# Autodesk Inventor assembly: !drive-pod-back-left
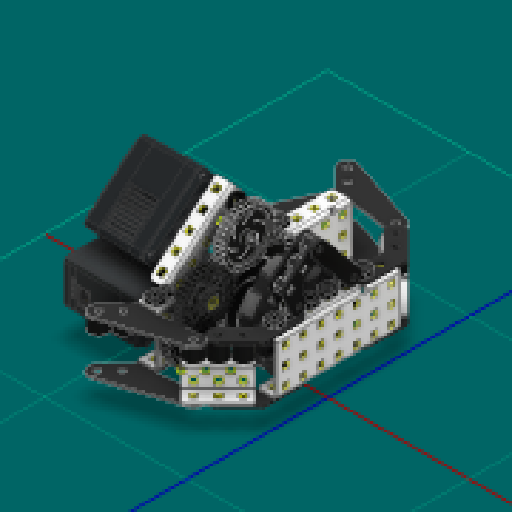
[picture p0: Inventor's stored thumbnail of the model, 512x512]
Saved by Autodesk Inventor 2025 (Build 290162000, 162)
## iProperties
Created: 2024-08-10
Part Number: !drive-pod-back-left
Document SubType Name: Assembly
Designer: averey
Author: averey
## Documents named in this file (25)
- C:\Users\avere\rbp_cad\atlas\chassis\drive-pod-back-left\!drive-pod-back-left.iam
- C:\Users\avere\rbp_cad\atlas\chassis\drive-pod-back-left\LS Pillow Bearing Block-back-left.ipt
- C:\Users\avere\rbp_cad\atlas\chassis\drive-pod-back-left\gearbox-support-gusset-back-left.ipt
- C:\Users\avere\rbp_cad\atlas\chassis\drive-pod-back-left\gearbox-gusset-back-left.ipt
- C:\Users\avere\rbp_cad\atlas\chassis\drive-pod-back-left\Bearing Flat Low Profile-back-left.ipt
- C:\Users\avere\rbp_cad\atlas\chassis\drive-pod-back-left\Alu Angle 1x1x5-back-left.ipt
- C:\Users\avere\rbp_cad\atlas\chassis\drive-pod-back-left\SteelM-StarS-back-left.iam
- C:\Users\avere\rbp_cad\atlas\chassis\drive-pod-back-left\V5 Motor (5.5W)-back-left.ipt
- C:\Users\avere\rbp_cad\atlas\chassis\drive-pod-back-left\LS 36T Gear-back-left.ipt
- C:\Users\avere\rbp_cad\atlas\chassis\drive-pod-back-left\LS 60T Gear-back-left.ipt
- C:\Users\avere\rbp_cad\atlas\chassis\drive-pod-back-left\2.75 Omni AS, No Insert-back-left.iam
- C:\Users\avere\rbp_cad\atlas\chassis\drive-pod-back-left\LS 12T Gear-back-left.ipt
- C:\Users\avere\rbp_cad\atlas\chassis\drive-pod-back-left\half_cut_36t-back-left.ipt
- C:\Users\avere\rbp_cad\atlas\chassis\drive-pod-back-left\elbow-gusset-back-left.ipt
- C:\Users\avere\rbp_cad\atlas\chassis\drive-pod-back-left\Alu C 1x2x1x3-back-left.ipt
- C:\Users\avere\rbp_cad\atlas\chassis\drive-pod-back-left\join-gusset_offset-back-left.ipt
- C:\Users\avere\rbp_cad\VEX-CAD-Inventor-1.41\Motion\Spacers\Spacer Nylon .500 OD\NSpacer Black .500 OD x .500.ipt
- C:\Users\avere\rbp_cad\VEX-CAD-Inventor-1.41\Motion\Spacers\Spacer Nylon .500 OD.ipt
- C:\Users\avere\rbp_cad\VEX-CAD-Inventor-1.41\Motion\Spacers\Spacer Nylon .500 OD\NSpacer Black .500 OD x .375.ipt
- C:\Users\avere\rbp_cad\VEX-CAD-Inventor-1.41\Structure\C Channel\Aluminum 1x3x1\Alu C 1x3x1x7.ipt
- C:\Users\avere\rbp_cad\VEX-CAD-Inventor-1.41\Structure\C Channel\Aluminum 1x3x1\Alu C 1x3x1x11.ipt
- C:\Users\avere\rbp_cad\atlas\chassis\drive-pod-back-right\join-gusset_offset-back-left-back-right.ipt
- C:\Users\avere\rbp_cad\VEX-CAD-Inventor-1.41\Structure\Standoff\Standoff 1.25.ipt
- C:\Users\avere\rbp_cad\VEX-CAD-Inventor-1.41\Motion\Spacers\Spacer Nylon .375 OD\NSpacer .375 OD x .125.ipt
- C:\Users\avere\rbp_cad\VEX-CAD-Inventor-1.41\Motion\Spacers\Spacer Nylon .375 OD.ipt
## Components (44 placed, 22 different names)
1. LS Pillow Bearing Block-back-left:1 — Mate:7, Insert:11
2. LS Pillow Bearing Block-back-left:2 — Insert:9, Mate:8
3. gearbox-support-gusset-back-left:1 — Insert:9
4. gearbox-gusset-back-left:1 — Mate:7, Mate:9
5. gearbox-support-gusset-back-left:2 — Mate:8
6. gearbox-gusset-back-left:2 — Insert:11
7. Bearing Flat Low Profile-back-left:1 — Mate:9
8. LS Pillow Bearing Block-back-left:3 — Insert:17, Insert:18
9. LS Pillow Bearing Block-back-left:4 — Insert:16
10. Alu Angle 1x1x5-back-left:1 — Insert:16, Mate:12, Mate:13, Mate:22, Insert:31, Insert:30, Insert:32
11. gearbox-gusset-back-left:3 — Mate:12, Insert:17
12. gearbox-gusset-back-left:4 — Mate:13, Insert:18
13. SteelM-StarS-back-left:1 [sub-assembly] — Insert:51, Mate:33
14. V5 Motor (5.5W)-back-left:1 — Mate:22, Insert:31
15. LS 36T Gear-back-left:1 — Insert:29
16. LS 60T Gear-back-left:1 — Insert:28, Mate:21, Insert:53
17. 2.75 Omni AS, No Insert-back-left:1 [sub-assembly] — Insert:28, Mate:21
18. LS 12T Gear-back-left:1 — Insert:29
19. half_cut_36t-back-left:1 — Insert:30
20. LS 36T Gear-back-left:2 — Insert:32
21. elbow-gusset-back-left:1 — Mate:25, Insert:35, Insert:45, Mate:28
22. Alu C 1x2x1x3-back-left:1 — Mate:25, Insert:35, Insert:38, Insert:41
23. elbow-gusset-back-left:2 — Insert:39, Insert:40
24. join-gusset_offset-back-left:1 — Insert:43, Insert:46
25. join-gusset_offset-back-left:2 — Insert:38, Insert:50, Mate:32
26. NSpacer Black .500 OD x .500:1 — Insert:39
27. NSpacer Black .500 OD x .500:2 — Insert:40
28. NSpacer Black .500 OD x .375:3 — Insert:41
29. NSpacer Black .500 OD x .375:4 — Insert:43
30. NSpacer Black .500 OD x .375:5 — Insert:46
31. Alu C 1x2x1x3-back-left:2 — Insert:39, Mate:25, Insert:41, Insert:42, Insert:54, Insert:55
32. elbow-gusset-back-left:3 — Insert:39, Mate:25, Insert:47, Mate:30
33. NSpacer Black .500 OD x .500:6 — Insert:41
34. NSpacer Black .500 OD x .500:7 — Insert:42
35. elbow-gusset-back-left:4 — Insert:48, Mate:29
36. Alu C 1x3x1x7:1 — Insert:45, Mate:28, Insert:47, Insert:48, Mate:29, Mate:30
37. Alu C 1x3x1x11:1 — Insert:50, Mate:32, Insert:51, Mate:33, Insert:53, Mate:34, Insert:59, Mate:35
38. join-gusset_offset-back-left-back-right:1 — Insert:54, Mate:34, Insert:56, Insert:57
39. NSpacer Black .500 OD x .375:8 — Insert:57
40. NSpacer Black .500 OD x .375:9 — Insert:56
41. NSpacer Black .500 OD x .375:10 — Insert:55
42. Standoff 1.25:1
43. NSpacer .375 OD x .125:1 — Insert:60
44. join-gusset_offset-back-left-back-right:2 — Insert:59, Mate:35, Insert:60
## Relationships (49: Insert 33, Mate 16)
- Insert:9: LS Pillow Bearing Block-back-left:2 ↔ gearbox-support-gusset-back-left:1
- Mate:7: LS Pillow Bearing Block-back-left:1 ↔ gearbox-gusset-back-left:1
- Mate:8: LS Pillow Bearing Block-back-left:2 ↔ gearbox-support-gusset-back-left:2
- Insert:11: LS Pillow Bearing Block-back-left:1 ↔ gearbox-gusset-back-left:2
- Mate:9: gearbox-gusset-back-left:1 ↔ Bearing Flat Low Profile-back-left:1
- Insert:16: LS Pillow Bearing Block-back-left:4 ↔ Alu Angle 1x1x5-back-left:1
- Mate:12: Alu Angle 1x1x5-back-left:1 ↔ gearbox-gusset-back-left:3
- Insert:17 (1.5875 mm): LS Pillow Bearing Block-back-left:3 ↔ gearbox-gusset-back-left:3
- Mate:13: Alu Angle 1x1x5-back-left:1 ↔ gearbox-gusset-back-left:4
- Insert:18: LS Pillow Bearing Block-back-left:3 ↔ gearbox-gusset-back-left:4
- Mate:22: Alu Angle 1x1x5-back-left:1 ↔ V5 Motor (5.5W)-back-left:1
- Insert:31: Alu Angle 1x1x5-back-left:1 ↔ V5 Motor (5.5W)-back-left:1
- Insert:28 (19.05 mm): LS 60T Gear-back-left:1 ↔ 2.75 Omni AS, No Insert-back-left:1
- Mate:21: LS 60T Gear-back-left:1 ↔ 2.75 Omni AS, No Insert-back-left:1
- Insert:29: LS 36T Gear-back-left:1 ↔ LS 12T Gear-back-left:1
- Insert:30 (11.5094 mm): Alu Angle 1x1x5-back-left:1 ↔ half_cut_36t-back-left:1
- Insert:32 (12.7 mm): Alu Angle 1x1x5-back-left:1 ↔ LS 36T Gear-back-left:2
- Mate:25: elbow-gusset-back-left:1 ↔ Alu C 1x2x1x3-back-left:1
- Insert:35: elbow-gusset-back-left:1 ↔ Alu C 1x2x1x3-back-left:1
- Insert:38: Alu C 1x2x1x3-back-left:1 ↔ join-gusset_offset-back-left:2
- Insert:39: elbow-gusset-back-left:2 ↔ NSpacer Black .500 OD x .500:1
- Insert:40: elbow-gusset-back-left:2 ↔ NSpacer Black .500 OD x .500:2
- Insert:41: Alu C 1x2x1x3-back-left:1 ↔ NSpacer Black .500 OD x .375:3
- Insert:43: join-gusset_offset-back-left:1 ↔ NSpacer Black .500 OD x .375:4
- Insert:39: Alu C 1x2x1x3-back-left:2 ↔ elbow-gusset-back-left:3
- Mate:25: Alu C 1x2x1x3-back-left:2 ↔ elbow-gusset-back-left:3
- Insert:41: Alu C 1x2x1x3-back-left:2 ↔ NSpacer Black .500 OD x .500:6
- Insert:42: Alu C 1x2x1x3-back-left:2 ↔ NSpacer Black .500 OD x .500:7
- Insert:45: elbow-gusset-back-left:1 ↔ Alu C 1x3x1x7:1
- Insert:46: join-gusset_offset-back-left:1 ↔ NSpacer Black .500 OD x .375:5
- Mate:28: elbow-gusset-back-left:1 ↔ Alu C 1x3x1x7:1
- Insert:47: elbow-gusset-back-left:3 ↔ Alu C 1x3x1x7:1
- Insert:48: elbow-gusset-back-left:4 ↔ Alu C 1x3x1x7:1
- Mate:29: elbow-gusset-back-left:4 ↔ Alu C 1x3x1x7:1
- Mate:30: elbow-gusset-back-left:3 ↔ Alu C 1x3x1x7:1
- Insert:50: join-gusset_offset-back-left:2 ↔ Alu C 1x3x1x11:1
- Mate:32: join-gusset_offset-back-left:2 ↔ Alu C 1x3x1x11:1
- Insert:51: SteelM-StarS-back-left:1 ↔ Alu C 1x3x1x11:1
- Mate:33: SteelM-StarS-back-left:1 ↔ Alu C 1x3x1x11:1
- Insert:53 (0.3969 mm): LS 60T Gear-back-left:1 ↔ Alu C 1x3x1x11:1
- Insert:54 (9.525 mm): Alu C 1x2x1x3-back-left:2 ↔ join-gusset_offset-back-left-back-right:1
- Mate:34: Alu C 1x3x1x11:1 ↔ join-gusset_offset-back-left-back-right:1
- Insert:55: Alu C 1x2x1x3-back-left:2 ↔ NSpacer Black .500 OD x .375:10
- Insert:56: join-gusset_offset-back-left-back-right:1 ↔ NSpacer Black .500 OD x .375:9
- Insert:57: join-gusset_offset-back-left-back-right:1 ↔ NSpacer Black .500 OD x .375:8
- [Insert]: Standoff 1.25:1 ↔ NSpacer .375 OD x .125:1
- Insert:59: Alu C 1x3x1x11:1 ↔ join-gusset_offset-back-left-back-right:2
- Mate:35: Alu C 1x3x1x11:1 ↔ join-gusset_offset-back-left-back-right:2
- Insert:60: NSpacer .375 OD x .125:1 ↔ join-gusset_offset-back-left-back-right:2
